# Autodesk Inventor assembly: MotionBaseGeneric
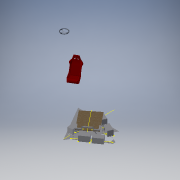
[picture p0: Inventor's stored thumbnail of the model, 180x180]
Saved by Autodesk Inventor 2016 (Build 200138000, 138)
## iProperties
Created: 2016-02-02
Part Number: MotionBaseGeneric
Document SubType Name: Assembly
Designer: tuttlem
math: 0.146 in
Author: tuttlem
## Documents named in this file (22)
- C:\Users\cutrones\Desktop\MotionBase\CAD\MotionBaseCAD\MotionBaseGeneric.iam
- C:\Users\cutrones\Desktop\MotionBase\CAD\MotionBaseCAD\Platform.ipt
- C:\Users\cutrones\Desktop\MotionBase\CAD\MotionBaseCAD\BasePlatform.ipt
- C:\Users\cutrones\Desktop\MotionBase\CAD\MotionBaseCAD\Rod.ipt
- C:\Users\cutrones\Desktop\MotionBase\CAD\MotionBaseCAD\Rod_MIR.ipt
- C:\Users\cutrones\Desktop\MotionBase\CAD\MotionBaseCAD\arm.ipt
- C:\Users\cutrones\Desktop\MotionBase\CAD\MotionBaseCAD\Bearing.ipt
- C:\Users\cutrones\Desktop\MotionBase\CAD\MotionBaseCAD\siege.ipt
- C:\Users\cutrones\Desktop\MotionBase\CAD\MotionBaseCAD\Sparco Volante wheel.ipt
- C:\Users\cutrones\Desktop\MotionBase\CAD\MotionBaseCAD\TopPlatform.ipt
- C:\Users\cutrones\Desktop\MotionBase\CAD\MotionBaseCAD\Side Rail.ipt
- C:\Users\cutrones\Desktop\MotionBase\CAD\MotionBaseCAD\Front Rail.ipt
- C:\Users\cutrones\Desktop\MotionBase\CAD\MotionBaseCAD\Imported Components\WGA-50M-080-H1\WGA-50M-080-H1.ipt
- C:\Users\cutrones\Desktop\MotionBase\CAD\MotionBaseCAD\Motor4.ipt
- C:\Users\cutrones\Desktop\MotionBase\CAD\MotionBaseCAD\GearShaft.ipt
- C:\Users\cutrones\Desktop\MotionBase\CAD\MotionBaseCAD\Triangle.ipt
- C:\Users\cutrones\Desktop\MotionBase\CAD\MotionBaseCAD\00 - Pedalier CSP V2.iam
- C:\Users\cutrones\Desktop\MotionBase\CAD\MotionBaseCAD\1inSquareSupport2.ipt
- C:\Users\cutrones\Desktop\MotionBase\CAD\MotionBaseCAD\1inSquareSupportOut.ipt
- C:\Users\cutrones\Desktop\MotionBase\CAD\MotionBaseCAD\corner plate.ipt
- U:\MotorCovers\RightCover\RightCover.iam
- C:\Users\cutrones\Desktop\MotionBase\CAD\MotionBaseCAD\MotorCovers\LeftCover\LeftMotorCover.iam
## Components (69 placed, 21 different names)
1. Platform:1 — Wood To Metal, Wood To Back, Mate:192, Mate:193, Mate:194, Mate:195, Mate:196, Mate:197, Mate:198
2. seat — Angle:9, Mate:72
3. Sparco Volante wheel:1
4. TopPlatform:1 — Wood To Metal, Wood To Back, Angle:8, Seat To Left, Mate:75, Mate:76, Flush:24, Flush:25, Flush:26, Flush:27, Mate:77, Flush:29, Flush:30, Mate:78, Flush:31, Flush:32, Angle:19, Mate:185, Flush:72, Angle:20, Mate:200
5. Side Rail:1 — Mate:75, Flush:24, Flush:26
6. Side Rail:2 — Mate:76, Flush:25, Flush:27
7. Front Rail:1 — Mate:77, Flush:29, Flush:30, Mate:186
8. Front Rail:2 — Mate:78, Flush:31, Flush:32
9. 00 - Pedalier CSP V2:2 [sub-assembly]
10. GearShaft:2 — Mate:109, Flush:40, Flush:45, Mate:148, Mate:149, Flush:55
11. GearShaft:4 — Mate:111, Flush:42, Flush:45, Mate:146, Mate:147, Flush:54
12. BasePlatform:2
13. GearShaft:8 — Mate:152, Mate:153, Flush:57
14. GearShaft:9 — Mate:154, Mate:155, Flush:58
15. GearShaft:10 — Mate:156, Mate:157, Flush:59
16. GearShaft:11 — Mate:150, Mate:151, Flush:56
17. Triangle:1 — Mate:214, Mate:215, Mate:216, Mate:217
18. 00 - Pedalier CSP V2:3 [sub-assembly] — Mate:185, Flush:72, Mate:186
19. 1inSquareSupport2:1 — Mate:204, Flush:78, Flush:79
20. 1inSquareSupportOut:1 — Mate:203, Flush:75, Flush:80, Mate:212, Flush:214, Flush:216, Flush:218, Mate:222, Flush:220, Mate:226
21. 1inSquareSupport2:2 — Mate:205, Flush:77, Flush:83, Symmetry:7
22. 1inSquareSupport2:3 — Mate:206, Flush:76, Flush:81, Flush:222
23. 1inSquareSupportOut:2 — Mate:202, Flush:74, Flush:82, Flush:85, Flush:217, Mate:220, Mate:230
24. 1inSquareSupportOut:3 — Mate:201, Flush:73, Flush:84, Mate:207, Mate:213, Symmetry:7, Flush:219, Mate:224, Flush:221, Mate:228
25. corner plate:1 — Mate:207, Mate:208, Flush:85
26. corner plate:2 — Flush:213, Mate:212, Flush:214
27. corner plate:3 — Mate:213, Flush:215, Flush:216
28. RightCover:1 [sub-assembly] — Flush:217, Mate:219, Mate:220
29. RightCover:2 [sub-assembly] — Flush:218, Mate:221, Mate:222
30. RightCover:3 [sub-assembly] — Flush:219, Mate:223, Mate:224
31. LeftMotorCover:4 [sub-assembly] — Flush:221, Mate:227, Mate:228
32. LeftMotorCover:5 [sub-assembly] — Flush:222, Mate:229, Mate:230
33. LeftMotorCover:6 [sub-assembly] — Flush:220, Mate:225, Mate:226
34. Motor4:11 — Flush:52, Mate:129, Angle:16, Angle:17, Symmetry:3, Symmetry:4, Mate:219
35. Motor4:10 — Flush:52, Symmetry:3, Symmetry:4, Mate:229
36. Motor4:9 — Flush:53, Mate:130, Angle:16, Symmetry:6, Mate:223
37. Motor4:8 — Flush:53, Symmetry:6, Mate:227
38. Motor4:7 — Mate:96, Angle:17, Symmetry:2, Symmetry:5, Mate:221
39. Motor4:1 — Mate:79, Angle:10, Mate:80, Mate:91, Symmetry:2, Symmetry:5, Mate:225
40. Rod_MIR:1 — Mate:101, Mate:173, Flush:66
41. Rod_MIR:2 — Mate:99, Mate:174, Flush:67
42. Rod_MIR:3 — Mate:28, Mate:175, Flush:68
43. Rod_MIR:4 — Mate:29, Mate:176, Flush:69
44. Rod_MIR:5 — Mate:97, Mate:177, Flush:70
45. Rod_MIR:6 — Mate:32, Mate:178, Flush:71
46. Rod:1 — Mate:173, Flush:66, Mate:197
47. Rod:2 — Mate:174, Flush:67, Mate:192
48. Rod:3 — Mate:175, Flush:68, Mate:194
49. Rod:4 — Mate:176, Flush:69, Mate:195
50. Rod:5 — Mate:177, Flush:70, Mate:196
51. Rod:6 — Mate:178, Flush:71, Mate:193
52. arm:1 — Mate:146, Mate:147, Flush:54, Mate:168, Flush:61
53. arm:8 — Mate:156, Mate:157, Flush:59, Mate:171, Flush:64
54. arm:9 — Mate:150, Mate:151, Flush:56, Mate:170, Flush:63
55. arm:10 — Mate:154, Mate:155, Flush:58, Mate:172, Flush:65
56. arm:11 — Mate:148, Mate:149, Flush:55, Mate:169, Flush:62
57. arm:12 — Mate:152, Mate:153, Flush:57, Mate:167, Flush:60
58. Bearing:2 — Mate:101, Mate:172, Flush:65
59. Bearing:3 — Mate:97, Mate:167, Flush:60
60. Bearing:4 — Mate:32, Mate:168, Flush:61
61. Bearing:5 — Mate:29, Mate:171, Flush:64
62. Bearing:6 — Mate:28, Mate:170, Flush:63
63. Bearing:1 — Mate:99, Mate:169, Flush:62
64. WGA-50M-080-H1:8 — Mate:136, Mate:201, Flush:77
65. WGA-50M-080-H1:9 — Mate:135, Flush:73, Mate:205
66. WGA-50M-080-H1:10 — Mate:134, Mate:202, Flush:76
67. WGA-50M-080-H1:11 — Mate:133, Flush:74, Mate:206
68. WGA-50M-080-H1:1 — Mate:79, Angle:10, Mate:80, Mate:109, Flush:40, Mate:132, Flush:75, Flush:78
69. WGA-50M-080-H1:7 — Mate:111, Flush:42, Mate:131, Mate:203, Mate:204
## Relationships (189: Mate 106, Flush 64, Angle 13, Symmetry 6)
- Flush:10 (25.4 mm)
- Mate:28: Rod_MIR:3 ↔ Bearing:6
- Mate:29: Rod_MIR:4 ↔ Bearing:5
- Mate:32: Rod_MIR:6 ↔ Bearing:4
- Angle:7 (0 deg)
- Wood To Metal [Mate]: Platform:1 ↔ TopPlatform:1
- Wood To Back [Flush] (-101.6 mm): Platform:1 ↔ TopPlatform:1
- Angle:8 (0 deg): TopPlatform:1
- Seat To Left [Flush] (-101.6 mm): TopPlatform:1
- Angle:9 (0 deg): seat
- Mate:72: seat
- Mate:75: TopPlatform:1 ↔ Side Rail:1
- Mate:76: TopPlatform:1 ↔ Side Rail:2
- Flush:24: TopPlatform:1 ↔ Side Rail:1
- Flush:25: TopPlatform:1 ↔ Side Rail:2
- Flush:26: TopPlatform:1 ↔ Side Rail:1
- Flush:27: TopPlatform:1 ↔ Side Rail:2
- Mate:77: TopPlatform:1 ↔ Front Rail:1
- Flush:29: TopPlatform:1 ↔ Front Rail:1
- Flush:30: TopPlatform:1 ↔ Front Rail:1
- Mate:78: TopPlatform:1 ↔ Front Rail:2
- Flush:31: TopPlatform:1 ↔ Front Rail:2
- Flush:32: TopPlatform:1 ↔ Front Rail:2
- Mate:79: Motor4:1 ↔ WGA-50M-080-H1:1
- Angle:10 (180 deg): Motor4:1 ↔ WGA-50M-080-H1:1
- Mate:80: Motor4:1 ↔ WGA-50M-080-H1:1
- [Mate]: Motor4:7 ↔ WGA-50M-080-H1:7
- [Angle] (180 deg): Motor4:7 ↔ WGA-50M-080-H1:7
- [Mate]: Motor4:7 ↔ WGA-50M-080-H1:7
- Mate:91: Motor4:1
- Mate:96: Motor4:7
- Mate:97: Rod_MIR:5 ↔ Bearing:3
- Mate:99: Rod_MIR:2 ↔ Bearing:1
- Mate:101: Rod_MIR:1 ↔ Bearing:2
- Mate:109: GearShaft:2 ↔ WGA-50M-080-H1:1
- Flush:40 (-88.9 mm): GearShaft:2 ↔ WGA-50M-080-H1:1
- Mate:111: GearShaft:4 ↔ WGA-50M-080-H1:7
- Flush:42 (-88.9 mm): GearShaft:4 ↔ WGA-50M-080-H1:7
- Flush:45: GearShaft:2 ↔ GearShaft:4
- [Mate]: Motor4:8 ↔ WGA-50M-080-H1:8
- [Angle] (180 deg): Motor4:8 ↔ WGA-50M-080-H1:8
- [Mate]: Motor4:8 ↔ WGA-50M-080-H1:8
- [Mate]: Motor4:9 ↔ WGA-50M-080-H1:9
- [Angle] (180 deg): Motor4:9 ↔ WGA-50M-080-H1:9
- [Mate]: Motor4:9 ↔ WGA-50M-080-H1:9
- [Mate]: GearShaft:8 ↔ WGA-50M-080-H1:8
- [Flush] (-114.3 mm): GearShaft:8 ↔ WGA-50M-080-H1:8
- [Mate]: GearShaft:9 ↔ WGA-50M-080-H1:9
- [Flush] (-114.3 mm): GearShaft:9 ↔ WGA-50M-080-H1:9
- [Flush]: GearShaft:8 ↔ GearShaft:9
- [Mate]: Motor4:10 ↔ WGA-50M-080-H1:10
- [Angle] (180 deg): Motor4:10 ↔ WGA-50M-080-H1:10
- [Mate]: Motor4:10 ↔ WGA-50M-080-H1:10
- [Mate]: Motor4:11 ↔ WGA-50M-080-H1:11
- [Angle] (180 deg): Motor4:11 ↔ WGA-50M-080-H1:11
- [Mate]: Motor4:11 ↔ WGA-50M-080-H1:11
- [Mate]: GearShaft:10 ↔ WGA-50M-080-H1:10
- [Flush] (-114.3 mm): GearShaft:10 ↔ WGA-50M-080-H1:10
- [Mate]: GearShaft:11 ↔ WGA-50M-080-H1:11
- [Flush] (-114.3 mm): GearShaft:11 ↔ WGA-50M-080-H1:11
- [Flush]: GearShaft:10 ↔ GearShaft:11
- Flush:52: Motor4:11 ↔ Motor4:10
- Flush:53: Motor4:9 ↔ Motor4:8
- Mate:129: Motor4:11
- Mate:130: Motor4:9
- Mate:131: WGA-50M-080-H1:7
- Mate:132: WGA-50M-080-H1:1
- Mate:133: WGA-50M-080-H1:11
- Mate:134: WGA-50M-080-H1:10
- Mate:135: WGA-50M-080-H1:9
- Mate:136: WGA-50M-080-H1:8
- Angle:16 (120 deg): Motor4:11 ↔ Motor4:9
- Angle:17 (240 deg): Motor4:11 ↔ Motor4:7
- Mate:146: GearShaft:4 ↔ arm:1
- Mate:147: GearShaft:4 ↔ arm:1
- Flush:54: GearShaft:4 ↔ arm:1
- Mate:148: GearShaft:2 ↔ arm:11
- Mate:149: GearShaft:2 ↔ arm:11
- Flush:55: GearShaft:2 ↔ arm:11
- Mate:150: GearShaft:11 ↔ arm:9
- Mate:151: GearShaft:11 ↔ arm:9
- Flush:56: GearShaft:11 ↔ arm:9
- Mate:152: GearShaft:8 ↔ arm:12
- Mate:153: GearShaft:8 ↔ arm:12
- Flush:57: GearShaft:8 ↔ arm:12
- Mate:154: GearShaft:9 ↔ arm:10
- Mate:155: GearShaft:9 ↔ arm:10
- Flush:58: GearShaft:9 ↔ arm:10
- Mate:156: GearShaft:10 ↔ arm:8
- Mate:157: GearShaft:10 ↔ arm:8
- Flush:59: GearShaft:10 ↔ arm:8
- Symmetry:2: Motor4:7 ↔ Motor4:1
- Symmetry:3: Motor4:11 ↔ Motor4:10
- Mate:158 (762 mm)
- Mate:159 (762 mm)
- Mate:160 (762 mm)
- Angle:19 (180 deg): TopPlatform:1
- Mate:167: arm:12 ↔ Bearing:3
- Flush:60: arm:12 ↔ Bearing:3
- Mate:168: arm:1 ↔ Bearing:4
- Flush:61: arm:1 ↔ Bearing:4
- Mate:169: arm:11 ↔ Bearing:1
- Flush:62: arm:11 ↔ Bearing:1
- Mate:170: arm:9 ↔ Bearing:6
- Flush:63: arm:9 ↔ Bearing:6
- Mate:171: arm:8 ↔ Bearing:5
- Flush:64: arm:8 ↔ Bearing:5
- Mate:172: arm:10 ↔ Bearing:2
- Flush:65: arm:10 ↔ Bearing:2
- Mate:173: Rod_MIR:1 ↔ Rod:1
- Flush:66: Rod_MIR:1 ↔ Rod:1
- Mate:174: Rod_MIR:2 ↔ Rod:2
- Flush:67: Rod_MIR:2 ↔ Rod:2
- Mate:175: Rod_MIR:3 ↔ Rod:3
- Flush:68: Rod_MIR:3 ↔ Rod:3
- Mate:176: Rod_MIR:4 ↔ Rod:4
- Flush:69: Rod_MIR:4 ↔ Rod:4
- Mate:177: Rod_MIR:5 ↔ Rod:5
- Flush:70: Rod_MIR:5 ↔ Rod:5
- Mate:178: Rod_MIR:6 ↔ Rod:6
- Flush:71: Rod_MIR:6 ↔ Rod:6
- Mate:185: TopPlatform:1 ↔ 00 - Pedalier CSP V2:3
- Flush:72: TopPlatform:1 ↔ 00 - Pedalier CSP V2:3
- Mate:186 (12.7 mm): Front Rail:1 ↔ 00 - Pedalier CSP V2:3
- Mate:190
- Mate:192: Platform:1 ↔ Rod:2
- Mate:193: Platform:1 ↔ Rod:6
- Mate:194: Platform:1 ↔ Rod:3
- Mate:195: Platform:1 ↔ Rod:4
- Mate:196: Platform:1 ↔ Rod:5
- Mate:197: Platform:1 ↔ Rod:1
- Mate:198: Platform:1
- Mate:199
- Angle:20 (0 deg): TopPlatform:1
- Mate:200 (-101.6 mm): TopPlatform:1
- Mate:201: 1inSquareSupportOut:3 ↔ WGA-50M-080-H1:8
- Flush:73 (-3.6957 mm): 1inSquareSupportOut:3 ↔ WGA-50M-080-H1:9
- Mate:202: 1inSquareSupportOut:2 ↔ WGA-50M-080-H1:10
- Flush:74 (-3.6957 mm): 1inSquareSupportOut:2 ↔ WGA-50M-080-H1:11
- Mate:203: 1inSquareSupportOut:1 ↔ WGA-50M-080-H1:7
- Flush:75 (-3.6957 mm): 1inSquareSupportOut:1 ↔ WGA-50M-080-H1:1
- Mate:204: 1inSquareSupport2:1 ↔ WGA-50M-080-H1:7
- Mate:205: 1inSquareSupport2:2 ↔ WGA-50M-080-H1:9
- Mate:206: 1inSquareSupport2:3 ↔ WGA-50M-080-H1:11
- Flush:76 (-3.6957 mm): 1inSquareSupport2:3 ↔ WGA-50M-080-H1:10
- Flush:77 (-3.6957 mm): 1inSquareSupport2:2 ↔ WGA-50M-080-H1:8
- Flush:78 (-3.6957 mm): 1inSquareSupport2:1 ↔ WGA-50M-080-H1:1
- Symmetry:4: Motor4:11 ↔ Motor4:10
- Symmetry:5: Motor4:7 ↔ Motor4:1
- Symmetry:6: Motor4:9 ↔ Motor4:8
- Flush:79 (-635 mm): 1inSquareSupport2:1
- Flush:80 (-711.2 mm): 1inSquareSupportOut:1
- Flush:81 (-635 mm): 1inSquareSupport2:3
- Flush:82 (-711.2 mm): 1inSquareSupportOut:2
- Flush:83 (-635 mm): 1inSquareSupport2:2
- Flush:84 (-711.2 mm): 1inSquareSupportOut:3
- Mate:207: 1inSquareSupportOut:3 ↔ corner plate:1
- Mate:208: corner plate:1
- Flush:85: 1inSquareSupportOut:2 ↔ corner plate:1
- Flush:213: corner plate:2
- Mate:212: 1inSquareSupportOut:1 ↔ corner plate:2
- Flush:214: 1inSquareSupportOut:1 ↔ corner plate:2
- Mate:213: 1inSquareSupportOut:3 ↔ corner plate:3
- Flush:215: corner plate:3
- Flush:216: 1inSquareSupportOut:1 ↔ corner plate:3
- Mate:214: Triangle:1
- Mate:215: Triangle:1
- Mate:216: Triangle:1
- Mate:217: Triangle:1
- Mate:218
- Symmetry:7: 1inSquareSupport2:2 ↔ 1inSquareSupportOut:3
- Flush:217: 1inSquareSupportOut:2 ↔ RightCover:1
- Mate:219 (25.4 mm): RightCover:1 ↔ Motor4:11
- Mate:220: 1inSquareSupportOut:2 ↔ RightCover:1
- Flush:218: 1inSquareSupportOut:1 ↔ RightCover:2
- Mate:221 (25.4 mm): RightCover:2 ↔ Motor4:7
- Mate:222: 1inSquareSupportOut:1 ↔ RightCover:2
- Flush:219: 1inSquareSupportOut:3 ↔ RightCover:3
- Mate:223 (25.4 mm): RightCover:3 ↔ Motor4:9
- Mate:224: 1inSquareSupportOut:3 ↔ RightCover:3
- Flush:220: 1inSquareSupportOut:1 ↔ LeftMotorCover:6
- Mate:225 (25.4 mm): LeftMotorCover:6 ↔ Motor4:1
- Mate:226: 1inSquareSupportOut:1 ↔ LeftMotorCover:6
- Flush:221: 1inSquareSupportOut:3 ↔ LeftMotorCover:4
- Mate:227 (25.4 mm): LeftMotorCover:4 ↔ Motor4:8
- Mate:228: 1inSquareSupportOut:3 ↔ LeftMotorCover:4
- Flush:222: 1inSquareSupport2:3 ↔ LeftMotorCover:5
- Mate:229 (25.4 mm): LeftMotorCover:5 ↔ Motor4:10
- Mate:230: 1inSquareSupportOut:2 ↔ LeftMotorCover:5
## Named parameters: d173_d169 = 0 mm, d174_d171 = 180 deg, d175_d172 = 0 mm, GearShaftL = 127 mm, d229_GearShaftL = 152.4 mm, d230_d216 = 0 mm, d231_d217 = -114.3 mm, d232_d220 = 0 mm, d233_d221 = -114.3 mm, d234_d226 = 0 mm, d236_d169 = 0 mm, d237_d171 = 180 deg, d238_d172 = 0 mm, d239_d173_d169 = 0 mm, d240_d174_d171 = 180 deg, d241_d175_d172 = 0 mm, d242_GearShaftL = 152.4 mm, d243_d216 = 0 mm, d244_d217 = -114.3 mm, d245_d220 = 0 mm, d246_d221 = -114.3 mm, d247_d226 = 0 mm, d249_d169 = 0 mm, d250_d171 = 180 deg, d251_d172 = 0 mm, d252_d173_d169 = 0 mm, d253_d174_d171 = 180 deg, d254_d175_d172 = 0 mm, math = 3.6957 mm, L = 1270 mm, L2 = 1422.4 mm
